# Autodesk Inventor assembly: Assembly_Total
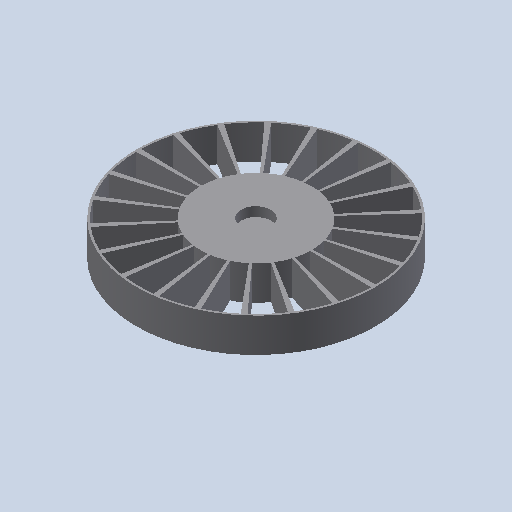
[picture p0: Inventor's stored thumbnail of the model, 512x512]
Saved by Autodesk Inventor 2022 (Build 260153000, 153)
## iProperties
Created: 2023-03-06
Part Number: Assembly_Total
Document SubType Name: Assembly
Designer: zarek
Author: zarek
## Documents named in this file (4)
- C:\Users\zarek\OneDrive\Desktop\Random New Stuff\SPB\Rotational_Piece_2.iam
- C:\Users\zarek\OneDrive\Desktop\Random New Stuff\SPB\GrabCad Parts\Stepper 28BYJ48.ipt
- C:\Users\zarek\OneDrive\Desktop\Random New Stuff\SPB\Capsule_Design_Revamp.ipt
- C:\Users\zarek\OneDrive\Desktop\Random New Stuff\SPB\Motor_Key_Cross.ipt
## Components (3 placed, 3 different names)
1. Stepper 28BYJ48:1 — Rigid:1
2. Capsule_Design_Revamp:1 — Mate:1, Mate:2, Mate:3
3. Motor_Key_Cross:1 — Rigid:1, Mate:1, Mate:2, Mate:3
## Relationships (4: Mate 3, WeldJoint 1)
- Rigid:1 [WeldJoint]: Stepper 28BYJ48:1 ↔ Motor_Key_Cross:1
- Mate:1: Capsule_Design_Revamp:1 ↔ Motor_Key_Cross:1
- Mate:2 (0.1 mm): Capsule_Design_Revamp:1 ↔ Motor_Key_Cross:1
- Mate:3 (0.1 mm): Capsule_Design_Revamp:1 ↔ Motor_Key_Cross:1
